# Autodesk Inventor assembly: C60-FW (CATALOG MODEL)
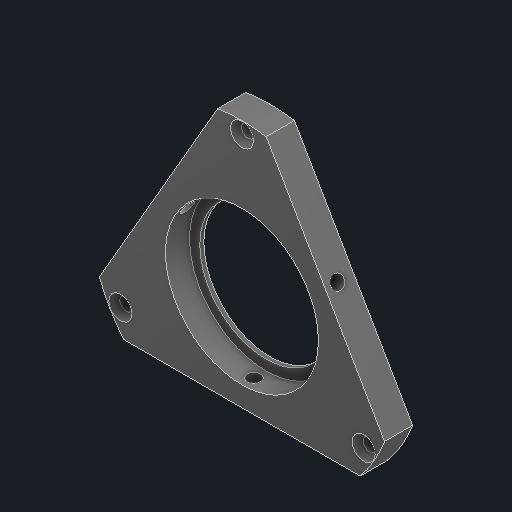
[picture p0: Inventor's stored thumbnail of the model, 512x512]
Saved by Autodesk Inventor 2026 (Build 300175000, 175)
## iProperties
Created: 2020-09-02
Part Number: C60-FW (CATALOG MODEL)
Material: Generic
Description: STEP AP214
Document SubType Name: Modeling
Designer: FiolkaLab
Density: 1 g/cm^3
Appearance: Default
Company: Microsoft
Title: C60-FW.STEP
Author: Aaron
Revision Number: ANY
Sending System: SolidWorks 2020
Preprocessor: SwSTEP 2.0
## Documents named in this file (4)
- **C:\Users\FiolkaLab\Desktop\Muaaz Rotation\Filter Wheel with Adapters.iam*LocalDocs*xAaaaqddaAaaaaaaaAaaaqwdlMc*C60-FW (CATALOG MODEL).ipt
- C:\Users\FiolkaLab\Desktop\Muaaz Rotation\Filter Wheel with Adapters.iam
- C:\Users\FiolkaLab\Desktop\Muaaz Rotation\FW-1000-8 with Holes.ipt
- C:\Users\FiolkaLab\Desktop\Muaaz Rotation\C60-FW (CATALOG MODEL).STEP
## Components (3 placed, 2 different names)
1. FW-1000-8 with Holes:1 — Mate:1, Mate:2, Mate:3, Mate:4
2. C60-FW (CATALOG MODEL):1 — Mate:1, Mate:2
3. C60-FW (CATALOG MODEL):2 — Mate:3, Mate:4
## Relationships (4: Mate 4)
- Mate:1: FW-1000-8 with Holes:1 ↔ C60-FW (CATALOG MODEL):1
- Mate:2: FW-1000-8 with Holes:1 ↔ C60-FW (CATALOG MODEL):1
- Mate:3: FW-1000-8 with Holes:1 ↔ C60-FW (CATALOG MODEL):2
- Mate:4: FW-1000-8 with Holes:1 ↔ C60-FW (CATALOG MODEL):2
